# Autodesk Inventor assembly: full
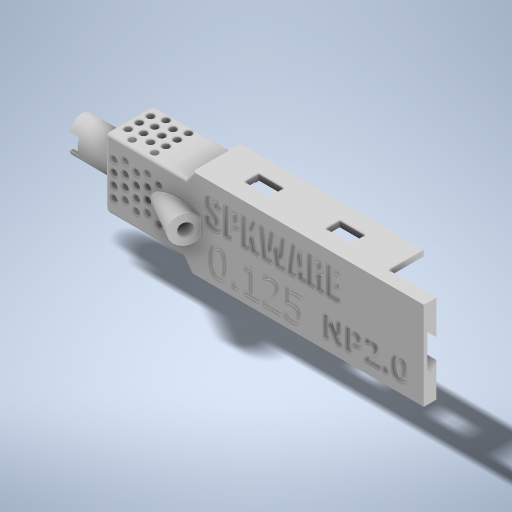
[picture p0: Inventor's stored thumbnail of the model, 512x512]
Saved by Autodesk Inventor 2023.3 (Build 273359000, 359)
## iProperties
RuleStatus: InUse
Created: 2023-03-21
Part Number: full
Document SubType Name: Assembly
Designer: joao
Author: joao
## Documents named in this file (11)
- X:\chronic_holder\NP2\np2_full_assembly.iam
- C:\Users\joao\lib\np_holder\NP2\probe\Neuropixels_20_metal cap_NPM_FLEX_01-01-009.iam
- X:\chronic_holder\NP2\1_main_chassis\np2_main_chassis.ipt
- X:\chronic_holder\NP2\2_cap\cap_no_headstage\np2_cap_no_headstage.ipt
- X:\chronic_holder\NP2\3_stereotax_holder\np2_stereotax_holder_part1.ipt
- X:\chronic_holder\NP2\3_stereotax_holder\np2_stereotax_holder_part2.ipt
- X:\chronic_holder\NP2\2_cap\cap_open_top\np2_cap_open_top.ipt
- X:\chronic_holder\NP2\2_cap\cap_with_headstage\np2_cap_with_headstage.ipt
- X:\chronic_holder\NP2\2_cap\cap_open_top\np2_headstage_box.ipt
- X:\chronic_holder\NP2\2_cap\cap_open_top\np2_headstage_box_v2.ipt
- X:\chronic_holder\NP2\2_cap\cap_with_headstage\top_enclosure.ipt
## Components (10 placed, 10 different names)
1. Neuropixels_20_metal cap_NPM_FLEX_01-01-009:1 [sub-assembly]
2. np2_main_chassis:1 — Flush:1, Flush:2, Flush:3, Flush:4
3. np2_cap_no_headstage:1
4. np2_stereotax_holder_part1:1 — Flush:1
5. np2_stereotax_holder_part2:1 — Flush:2
6. np2_cap_open_top:1 — Flush:3
7. np2_cap_with_headstage:1 — Flush:4
8. np2_headstage_box:1
9. np2_headstage_box_v2:1
10. top_enclosure:1
## Relationships (4: Flush 4)
- Flush:1: np2_main_chassis:1 ↔ np2_stereotax_holder_part1:1
- Flush:2: np2_main_chassis:1 ↔ np2_stereotax_holder_part2:1
- Flush:3: np2_main_chassis:1 ↔ np2_cap_open_top:1
- Flush:4: np2_main_chassis:1 ↔ np2_cap_with_headstage:1
